# Autodesk Inventor assembly: Gertiebe
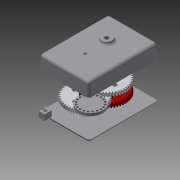
[picture p0: Inventor's stored thumbnail of the model, 180x180]
Saved by Autodesk Inventor 2014 (Build 180170000, 170)
## iProperties
Created: 2013-05-31
Part Number: Gertiebe
Document SubType Name: Assembly
Designer: hanse
Author: hanse
## Documents named in this file (7)
- C:\Users\Felix\Desktop\Beep\Hardware\GetriebeB\Gertiebe.iam
- C:\Users\Felix\Desktop\Beep\Hardware\GetriebeB\Gertiebe\Konstruktions-Assistent\Stirnräder3.iam
- C:\Users\Felix\Desktop\Beep\Hardware\GetriebeB\DoppelZahnrad.iam
- C:\Users\Felix\Desktop\Beep\Hardware\GetriebeB\GehäuseFront.ipt
- C:\Users\Felix\Desktop\Beep\Hardware\GetriebeB\GehäuseBack.ipt
- C:\Users\Felix\Desktop\Beep\Hardware\EE-SX1131.ipt
- C:\Users\Felix\Desktop\Beep\Hardware\GetriebeB\EncoderWheel2.ipt
## Components (8 placed, 6 different names)
1. Stirnräder:3 [sub-assembly] — Passend:1, Passend:2, Passend:5, Passend:6, Passend:8
2. DoppelZahnrad:1 [sub-assembly] — Passend:1, Passend:3, Passend:9
3. DoppelZahnrad:2 [sub-assembly] — Passend:2, Passend:8, Passend:10
4. DoppelZahnrad:3 [sub-assembly] — Passend:3, Passend:4, Passend:7, Passend:9
5. GehäuseFront:1 — Passend:4, Passend:5, Passend:6, Passend:7, Passend:11
6. GehäuseBack:1 — Passend:10
7. EE-SX1131:1
8. EncoderWheel2:1
## Relationships (11: Mate 11)
- Passend:1 [Mate] (15 mm): Stirnräder:3 ↔ DoppelZahnrad:1
- Passend:2 [Mate]: Stirnräder:3 ↔ DoppelZahnrad:2
- Passend:3 [Mate]: DoppelZahnrad:1 ↔ DoppelZahnrad:3
- Passend:4 [Mate]: DoppelZahnrad:3 ↔ GehäuseFront:1
- Passend:5 [Mate]: Stirnräder:3 ↔ GehäuseFront:1
- Passend:6 [Mate]: Stirnräder:3 ↔ GehäuseFront:1
- Passend:7 [Mate]: DoppelZahnrad:3 ↔ GehäuseFront:1
- Passend:8 [Mate]: Stirnräder:3 ↔ DoppelZahnrad:2
- Passend:9 [Mate]: DoppelZahnrad:1 ↔ DoppelZahnrad:3
- Passend:10 [Mate]: DoppelZahnrad:2 ↔ GehäuseBack:1
- Passend:11 [Mate]: GehäuseFront:1
